# Autodesk Inventor assembly: autobuoy_full
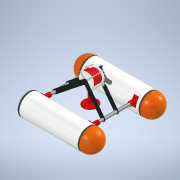
[picture p0: Inventor's stored thumbnail of the model, 180x180]
Saved by Autodesk Inventor 2020.2 (Build 242310000, 310)
## iProperties
Created: 2019-11-08
Part Number: autobuoy_full
Document SubType Name: Assembly
Designer: agmle
Mass: 22312 g
Surface Area: 36035.9 cm^2
Volume: 16913.6 cm^3
Density: 1.31918 g/cm^3
Author: agmle
## Documents named in this file (15)
- D:\projects\CreekFleet_AutoBuoy\Mechanical CAD\autobuoy_full.iam
- D:\projects\CreekFleet_AutoBuoy\Mechanical CAD\propulsion\drive_left.iam
- D:\projects\CreekFleet_AutoBuoy\Mechanical CAD\propulsion\drive_right.iam
- D:\projects\CreekFleet_AutoBuoy\Mechanical CAD\hull\hull_mid.ipt
- D:\projects\CreekFleet_AutoBuoy\Mechanical CAD\propulsion\onxp5510.ipt
- D:\projects\CreekFleet_AutoBuoy\Mechanical CAD\hull\forward_endcap.ipt
- D:\projects\CreekFleet_AutoBuoy\Mechanical CAD\hull\aft_right_endcap.ipt
- D:\projects\CreekFleet_AutoBuoy\Mechanical CAD\hull\aft_left_endcap.ipt
- D:\projects\CreekFleet_AutoBuoy\Mechanical CAD\hull\hull_seal.ipt
- D:\projects\CreekFleet_AutoBuoy\Mechanical CAD\hull\strut.iam
- D:\projects\CreekFleet_AutoBuoy\Mechanical CAD\station-keeping\winch.iam
- D:\projects\CreekFleet_AutoBuoy\Mechanical CAD\controls\buoy_mainboard.iam
- D:\projects\CreekFleet_AutoBuoy\Mechanical CAD\controls\pololu\g2-high-power-motor-driver-md31a.ipt
- D:\projects\CreekFleet_AutoBuoy\Mechanical CAD\controls\pololu\ACS711EX.ipt
- D:\projects\CreekFleet_AutoBuoy\Mechanical CAD\parameters.xlsx
## Components (20 placed, 13 different names)
1. strut:1 [sub-assembly] — Mate:11, Mate:13, Mate:14, Mate:18, Mate:19
2. strut:2 [sub-assembly] — Mate:12, Mate:15, Mate:16, Mate:17
3. winch:1 [sub-assembly] — Mate:17, Mate:18, Mate:19
4. onxp5510:1 — Tangent:6, Tangent:7, Flush:3, Mate:6
5. drive_left:1 [sub-assembly] — Mate:1, Mate:2, Tangent:10, Flush:1, Flush:2, Mate:6, Flush:5, Mate:20, Mate:21, Flush:7, Mate:22, Mate:23, Tangent:12, Angle:1
6. onxp5510:2 — Tangent:4, Tangent:5, Flush:3, Mate:5
7. drive_right:1 [sub-assembly] — Mate:3, Mate:4, Tangent:11, Flush:1, Flush:2, Mate:5, Flush:4
8. buoy_mainboard:1 [sub-assembly] — Mate:24, Angle:1, Mate:25
9. g2-high-power-motor-driver-md31a:1 — Mate:20, Mate:21, Flush:7
10. ACS711EX:1 — Mate:22, Mate:23, Tangent:12
11. hull_mid:2 — Tangent:6, Tangent:7, Insert:2, Tangent:9, Mate:1, Mate:2, Tangent:10, Insert:4, Mate:7, Mate:10, Mate:11, Mate:12, Mate:24
12. forward_endcap:2 — Insert:2, Mate:25
13. aft_left_endcap:1 — Insert:4, Flush:5
14. hull_seal:1 — Mate:7
15. hull_seal:2 — Mate:10, Mate:16
16. hull_mid:1 — Tangent:4, Tangent:5, Insert:1, Tangent:8, Insert:3, Mate:3, Mate:4, Tangent:11, Mate:8, Mate:9, Mate:13, Mate:15
17. forward_endcap:1 — Insert:1
18. aft_right_endcap:1 — Insert:3, Flush:4
19. hull_seal:3 — Mate:9
20. hull_seal:4 — Mate:8, Mate:14
## Relationships (45: Mate 25, Tangent 9, Flush 6, Insert 4, Angle 1)
- Tangent:4: onxp5510:2 ↔ hull_mid:1
- Tangent:5: onxp5510:2 ↔ hull_mid:1
- Tangent:6: onxp5510:1 ↔ hull_mid:2
- Tangent:7: onxp5510:1 ↔ hull_mid:2
- Insert:1: hull_mid:1 ↔ forward_endcap:1
- Insert:2: hull_mid:2 ↔ forward_endcap:2
- Tangent:8: hull_mid:1
- Tangent:9: hull_mid:2
- Insert:3: hull_mid:1 ↔ aft_right_endcap:1
- Mate:1: drive_left:1 ↔ hull_mid:2
- Mate:2: drive_left:1 ↔ hull_mid:2
- Tangent:10: drive_left:1 ↔ hull_mid:2
- Mate:3: drive_right:1 ↔ hull_mid:1
- Mate:4: drive_right:1 ↔ hull_mid:1
- Tangent:11: drive_right:1 ↔ hull_mid:1
- Flush:1: drive_left:1 ↔ drive_right:1
- Flush:2: drive_left:1 ↔ drive_right:1
- Flush:3: onxp5510:1 ↔ onxp5510:2
- Mate:5: onxp5510:2 ↔ drive_right:1
- Mate:6: onxp5510:1 ↔ drive_left:1
- Flush:4: drive_right:1 ↔ aft_right_endcap:1
- Insert:4: hull_mid:2 ↔ aft_left_endcap:1
- Flush:5: drive_left:1 ↔ aft_left_endcap:1
- Mate:7: hull_mid:2 ↔ hull_seal:1
- Mate:8: hull_mid:1 ↔ hull_seal:4
- Mate:9: hull_mid:1 ↔ hull_seal:3
- Mate:10: hull_mid:2 ↔ hull_seal:2
- Mate:11: strut:1 ↔ hull_mid:2
- Mate:12: strut:2 ↔ hull_mid:2
- Mate:13: strut:1 ↔ hull_mid:1
- Mate:14 (25.4 mm): strut:1 ↔ hull_seal:4
- Mate:15: strut:2 ↔ hull_mid:1
- Mate:16 (25.4 mm): strut:2 ↔ hull_seal:2
- Mate:17: strut:2 ↔ winch:1
- Mate:18: strut:1 ↔ winch:1
- Mate:19 (82.55 mm): strut:1 ↔ winch:1
- Mate:20: drive_left:1 ↔ g2-high-power-motor-driver-md31a:1
- Mate:21: drive_left:1 ↔ g2-high-power-motor-driver-md31a:1
- Flush:7: drive_left:1 ↔ g2-high-power-motor-driver-md31a:1
- Mate:22: drive_left:1 ↔ ACS711EX:1
- Mate:23: drive_left:1 ↔ ACS711EX:1
- Tangent:12: drive_left:1 ↔ ACS711EX:1
- Mate:24: buoy_mainboard:1 ↔ hull_mid:2
- Angle:1 (0 deg): drive_left:1 ↔ buoy_mainboard:1
- Mate:25 (101.6 mm): buoy_mainboard:1 ↔ forward_endcap:2
## Named parameters: hull_od = 219.075 mm, hull_id = 201.7268 mm, hull_wall = 8.6741 mm, hull_length = 609.6 mm, hull_spacing = 390.525 mm, impeller_od = 76.2 mm, impeller_height = 20 mm, impeller_clearance = 0.5 mm, impeller_shaft_id = 3.175 mm, impeller_shaft_od = 5.715 mm, impeller_shaft_support = 3.175 mm, impeller_num_vanes = 6, impeller_intake_od = 19.05 mm, impeller_vane_thick = 2 mm, impeller_vane_inner_rad = 3.175 mm, impeller_vane_outer_rad = 0.37206 mm, magnet_od = 5.95 mm, magnet_length = 10 mm, magnet_clearance = 0.25 mm, magnet_rad = 0.25 mm, magnet_circle_offset = 3.175 mm, motor_shaft_od = 12.7 mm, motor_shaft_length = 31.75 mm, motor_shaft_key = 3.048 mm
